# Autodesk Inventor assembly: Kit Frame 28x28 open front
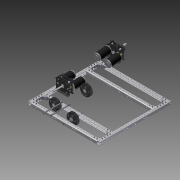
[picture p0: Inventor's stored thumbnail of the model, 180x180]
Saved by Autodesk Inventor 2013 (Build 170138000, 138)
## iProperties
Created: 2013-01-06
Part Number: Kit Frame 28x28 open front
Document SubType Name: Assembly
Designer: Nemo
Author: Nemo
## Documents named in this file (8)
- \\lmss\students\Robotics\CAD Files\COTS Parts\Kit Frame - AndyMark\Kit Frame 28x28.iam
- \\lmss\students\Robotics\CAD Files\COTS Parts\Kit Frame - AndyMark\Components\28x28 Side Rail sub.iam
- \\lmss\students\Robotics\CAD Files\COTS Parts\Kit Frame - AndyMark\Components\28x28 Side Rail Sub mirror.iam
- \\lmss\students\Robotics\CAD Files\COTS Parts\Kit Frame - AndyMark\Components\C Channel - FrontBack 28x28.ipt
- \\lmss\students\Robotics\CAD Files\COTS Parts\Gearboxes\VexPro 64 Single Stage Gearbox - Flanges Out.iam
- \\lmss\students\Robotics\CAD Files\COTS Parts\Wheels\VexPro VersaWheel 4in.ipt
- \\lmss\students\Robotics\CAD Files\COTS Parts\Fasteners\38-16 hexbolt x7000.ipt
- \\lmss\students\Robotics\CAD Files\COTS Parts\Bearings - VexPro\Flanged Bearing - 0.375in Round ID x 1.125in OD.ipt
## Components (20 placed, 7 different names)
1. C Channel - Cut-01:3 — Flush:5, Flush:6
2. C Channel - Cut-01:4 — Mate:3, Mate:4, Flush:6, Insert:1, Insert:2, Mate:5, Insert:3, Mate:6, Insert:4, Mate:7
3. 28x28 Side Rail sub:1 [sub-assembly] — Flush:7, Insert:1, Insert:11
4. 28x28 Side Rail Sub mirror:1 [sub-assembly] — Insert:3, Mate:6
5. 28x28 Side Rail sub:2 [sub-assembly] — Insert:4, Mate:7
6. 28x28 Side Rail Sub mirror:2 [sub-assembly] — Insert:2, Mate:5
7. VexPro 64 Single Stage Gearbox - Flanges Out:1 [sub-assembly]
8. VexPro 64 Single Stage Gearbox - Flanges Out:2 [sub-assembly]
9. VexPro VersaWheel 4in:6 — Insert:16, Insert:17
10. VexPro VersaWheel 4in:7 — Insert:12, Insert:13
11. VexPro VersaWheel 4in:8 — Insert:14, Insert:15
12. 38-16 hexbolt x7000:1 — Insert:11, Mate:8
13. 38-16 hexbolt x7000:2
14. 38-16 hexbolt x7000:3
15. Flanged Bearing - 0.375in Round ID x 1.125in OD:1 — Insert:12
16. Flanged Bearing - 0.375in Round ID x 1.125in OD:2 — Insert:13
17. Flanged Bearing - 0.375in Round ID x 1.125in OD:3 — Insert:15
18. Flanged Bearing - 0.375in Round ID x 1.125in OD:4 — Insert:14, Mate:8
19. Flanged Bearing - 0.375in Round ID x 1.125in OD:5 — Insert:17
20. Flanged Bearing - 0.375in Round ID x 1.125in OD:6 — Insert:16
## Relationships (20: Insert 11, Mate 6, Flush 3)
- Flush:5: C Channel - Cut-01:3
- Mate:3: C Channel - Cut-01:4
- Mate:4 (36.83 mm): C Channel - Cut-01:4
- Flush:6: C Channel - Cut-01:3 ↔ C Channel - Cut-01:4
- Flush:7: 28x28 Side Rail sub:1
- Insert:1: C Channel - Cut-01:4 ↔ 28x28 Side Rail sub:1
- Insert:2: C Channel - Cut-01:4 ↔ 28x28 Side Rail Sub mirror:2
- Mate:5: C Channel - Cut-01:4 ↔ 28x28 Side Rail Sub mirror:2
- Insert:3: C Channel - Cut-01:4 ↔ 28x28 Side Rail Sub mirror:1
- Mate:6: C Channel - Cut-01:4 ↔ 28x28 Side Rail Sub mirror:1
- Insert:4: C Channel - Cut-01:4 ↔ 28x28 Side Rail sub:2
- Mate:7: C Channel - Cut-01:4 ↔ 28x28 Side Rail sub:2
- Insert:11: 28x28 Side Rail sub:1 ↔ 38-16 hexbolt x7000:1
- Insert:12: VexPro VersaWheel 4in:7 ↔ Flanged Bearing - 0.375in Round ID x 1.125in OD:1
- Insert:13: VexPro VersaWheel 4in:7 ↔ Flanged Bearing - 0.375in Round ID x 1.125in OD:2
- Insert:14: VexPro VersaWheel 4in:8 ↔ Flanged Bearing - 0.375in Round ID x 1.125in OD:4
- Insert:15: VexPro VersaWheel 4in:8 ↔ Flanged Bearing - 0.375in Round ID x 1.125in OD:3
- Insert:16: VexPro VersaWheel 4in:6 ↔ Flanged Bearing - 0.375in Round ID x 1.125in OD:6
- Insert:17: VexPro VersaWheel 4in:6 ↔ Flanged Bearing - 0.375in Round ID x 1.125in OD:5
- Mate:8: 38-16 hexbolt x7000:1 ↔ Flanged Bearing - 0.375in Round ID x 1.125in OD:4
